# Autodesk Inventor assembly: Bumper Assembly4 (24x28 robot)
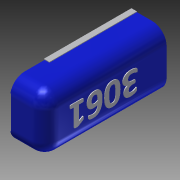
[picture p0: Inventor's stored thumbnail of the model, 180x180]
Saved by Autodesk Inventor 2013 (Build 170138000, 138)
## iProperties
Created: 2013-01-06
Part Number: Bumper Assembly4 (24x28 robot)
Document SubType Name: Assembly
Designer: Moses
Mass: 479.395 g
Surface Area: 4451.04 cm^2
Volume: 2087.03 cm^3
Density: 0.229702 g/cm^3
Author: Moses
## Documents named in this file (5)
- C:\Users\Moses\Documents\GitHub\frc2013CAD\Chassis\Bumpers\Bumper Assembly4 (24x28 robot).iam
- C:\Users\Moses\Documents\GitHub\frc2013CAD\Chassis\Bumpers\Bumper Wood Backing Part4 (24x28 robot).ipt
- C:\Users\Moses\Documents\GitHub\frc2013CAD\Chassis\Bumpers\Pool Noodle Part4 (24x28 robot).ipt
- C:\Users\Moses\Documents\GitHub\frc2013CAD\Chassis\Bumpers\Bumper Cover Part4 (24x28 robot).ipt
- C:\Users\Moses\Documents\GitHub\frc2013CAD\Chassis\Bumpers\Bumper Metal Edge Part4 (24x28 robot).ipt
## Components (6 placed, 4 different names)
1. Bumper Wood Backing Part4 (24x28 robot):1 — Flush:1, Flush:2, Tangent:2, Tangent:3, Tangent:4, Mate:1, Mate:2
2. Pool Noodle Part4 (24x28 robot):1 — Flush:1, Tangent:1, Tangent:2, Tangent:4, Tangent:5
3. Pool Noodle Part4 (24x28 robot):2 — Flush:2, Tangent:1, Tangent:3
4. Bumper Cover Part4 (24x28 robot):1 — Mate:1, Mate:2, Tangent:5, Mate:3, Mate:4, Flush:3, Mate:5, Mate:6, Flush:4
5. Bumper Metal Edge Part4 (24x28 robot):1 — Mate:3, Mate:4, Flush:3
6. Bumper Metal Edge Part4 (24x28 robot):2 — Mate:5, Mate:6, Flush:4
## Relationships (15: Mate 6, Tangent 5, Flush 4)
- Flush:1 (19.05 mm): Bumper Wood Backing Part4 (24x28 robot):1 ↔ Pool Noodle Part4 (24x28 robot):1
- Flush:2 (19.05 mm): Bumper Wood Backing Part4 (24x28 robot):1 ↔ Pool Noodle Part4 (24x28 robot):2
- Tangent:1: Pool Noodle Part4 (24x28 robot):1 ↔ Pool Noodle Part4 (24x28 robot):2
- Tangent:2: Bumper Wood Backing Part4 (24x28 robot):1 ↔ Pool Noodle Part4 (24x28 robot):1
- Tangent:3: Bumper Wood Backing Part4 (24x28 robot):1 ↔ Pool Noodle Part4 (24x28 robot):2
- Tangent:4: Bumper Wood Backing Part4 (24x28 robot):1 ↔ Pool Noodle Part4 (24x28 robot):1
- Mate:1: Bumper Wood Backing Part4 (24x28 robot):1 ↔ Bumper Cover Part4 (24x28 robot):1
- Mate:2: Bumper Wood Backing Part4 (24x28 robot):1 ↔ Bumper Cover Part4 (24x28 robot):1
- Tangent:5: Pool Noodle Part4 (24x28 robot):1 ↔ Bumper Cover Part4 (24x28 robot):1
- Mate:3: Bumper Cover Part4 (24x28 robot):1 ↔ Bumper Metal Edge Part4 (24x28 robot):1
- Mate:4: Bumper Cover Part4 (24x28 robot):1 ↔ Bumper Metal Edge Part4 (24x28 robot):1
- Flush:3: Bumper Cover Part4 (24x28 robot):1 ↔ Bumper Metal Edge Part4 (24x28 robot):1
- Mate:5: Bumper Cover Part4 (24x28 robot):1 ↔ Bumper Metal Edge Part4 (24x28 robot):2
- Mate:6: Bumper Cover Part4 (24x28 robot):1 ↔ Bumper Metal Edge Part4 (24x28 robot):2
- Flush:4: Bumper Cover Part4 (24x28 robot):1 ↔ Bumper Metal Edge Part4 (24x28 robot):2
